# Autodesk Inventor assembly: Synchronous Belts Transmission
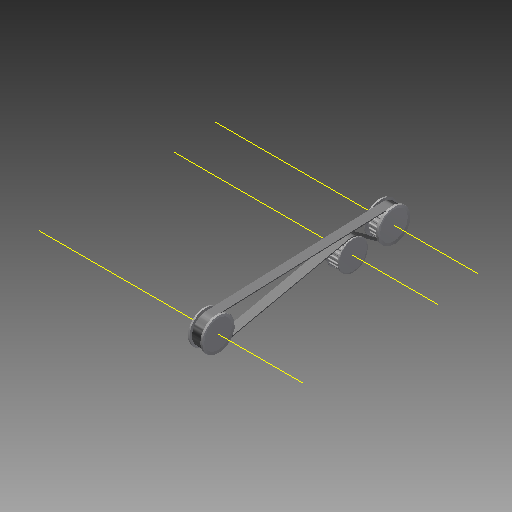
[picture p0: Inventor's stored thumbnail of the model, 512x512]
Saved by Autodesk Inventor 2019.4 (Build 234330000, 330)
## iProperties
Created: 2020-01-23
Part Number: Synchronous Belts Transmission
Document SubType Name: Assembly
Designer: admin
Mass: 107.181 g
Surface Area: 145.863 cm^2
Volume: 16.9594 cm^3
Density: 6.31987 g/cm^3
ClientObjectVersion: 1
Author: admin
## Documents named in this file (5)
- C:\Users\admin\Desktop\FRC 2020 Engineering\GitHub\7738-2020\Robot V2\Turret Columb Assembly\Turret Columb Assembly\Design Accelerator\Synchronous Belts Transmission7.iam
- C:\Users\admin\Desktop\FRC 2020 Engineering\GitHub\7738-2020\Robot V2\Turret Columb Assembly\Turret Columb Assembly\Design Accelerator\Synchronous Belt7.ipt
- C:\Users\admin\Desktop\FRC 2020 Engineering\GitHub\7738-2020\Robot V2\Turret Columb Assembly\Turret Columb Assembly\Design Accelerator\Synchronous Pulley17.ipt
- C:\Users\admin\Desktop\FRC 2020 Engineering\GitHub\7738-2020\Robot V2\Turret Columb Assembly\Turret Columb Assembly\Design Accelerator\Synchronous Pulley27.ipt
- C:\Users\admin\Desktop\FRC 2020 Engineering\GitHub\7738-2020\Robot V2\Turret Columb Assembly\Turret Columb Assembly\Design Accelerator\Synchronous Pulley31.ipt
## Components (4 placed, 4 different names)
1. Synchronous Belt:1 — Flush:1, Mate:1, Mate:2, Flush:2, Mate:3, Mate:4, Flush:3, Mate:5, Mate:6
2. Synchronous Pulley1:1 — Flush:1, Mate:1, Mate:2, Rotation:1, Rotation:2
3. Synchronous Pulley2:1 — Flush:2, Mate:3, Rotation:1, Mate:4
4. Synchronous Pulley3:1 — Flush:3, Mate:5, Rotation:2, Mate:6
## Relationships (11: Mate 6, Flush 3, RelateRotation 2)
- Flush:1: Synchronous Belt:1 ↔ Synchronous Pulley1:1
- Mate:1: Synchronous Belt:1 ↔ Synchronous Pulley1:1
- Mate:2: Synchronous Belt:1 ↔ Synchronous Pulley1:1
- Flush:2: Synchronous Belt:1 ↔ Synchronous Pulley2:1
- Mate:3: Synchronous Belt:1 ↔ Synchronous Pulley2:1
- Rotation:1 [RelateRotation] (1 ul): Synchronous Pulley1:1 ↔ Synchronous Pulley2:1
- Mate:4: Synchronous Belt:1 ↔ Synchronous Pulley2:1
- Flush:3: Synchronous Belt:1 ↔ Synchronous Pulley3:1
- Mate:5: Synchronous Belt:1 ↔ Synchronous Pulley3:1
- Rotation:2 [RelateRotation] (1 ul): Synchronous Pulley1:1 ↔ Synchronous Pulley3:1
- Mate:6: Synchronous Belt:1 ↔ Synchronous Pulley3:1
